# Autodesk Inventor assembly: Electronics Mount
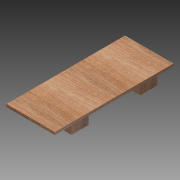
[picture p0: Inventor's stored thumbnail of the model, 180x180]
Saved by Autodesk Inventor 2014 (Build 180170000, 170)
## iProperties
Created: 2016-02-05
Part Number: Electronics Mount
Document SubType Name: Assembly
Designer: zoldberg
Author: zoldberg
## Documents named in this file (3)
- Z:\Nerds_1726\Models\2015-2016\Assemblies\Robot\Electronics Mount.iam
- Z:\Nerds_1726\Models\2015-2016\Parts\Robot\Electronics\LeftMountingBoard.ipt
- Z:\Nerds_1726\Models\2015-2016\Parts\Robot\Electronics\LeftMountingBoard2x4.ipt
## Components (3 placed, 2 different names)
1. LeftMountingBoard:1 — Flush:1, Flush:2, Flush:3, Flush:4, Mate:1, Mate:2
2. LeftMountingBoard2x4:1 — Flush:1, Flush:3, Mate:1
3. LeftMountingBoard2x4:2 — Flush:2, Flush:4, Mate:2
## Relationships (6: Flush 4, Mate 2)
- Flush:1: LeftMountingBoard:1 ↔ LeftMountingBoard2x4:1
- Flush:2: LeftMountingBoard:1 ↔ LeftMountingBoard2x4:2
- Flush:3 (76.2 mm): LeftMountingBoard:1 ↔ LeftMountingBoard2x4:1
- Flush:4 (76.2 mm): LeftMountingBoard:1 ↔ LeftMountingBoard2x4:2
- Mate:1: LeftMountingBoard:1 ↔ LeftMountingBoard2x4:1
- Mate:2: LeftMountingBoard:1 ↔ LeftMountingBoard2x4:2
